# Autodesk Inventor assembly: SailAssembly
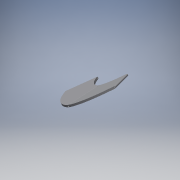
[picture p0: Inventor's stored thumbnail of the model, 180x180]
Saved by Autodesk Inventor 2018.3 (Build 223284000, 284)
## iProperties
Created: 2020-03-24
Part Number: SailAssembly
Document SubType Name: Assembly
Designer: ToreDenStore
Author: ToreDenStore
## Documents named in this file (2)
- C:\Users\ToreDenStore\Documents\Inventor\VAWT turbine sunfeather\SailAssembly.iam
- C:\Users\ToreDenStore\Documents\Inventor\VAWT turbine sunfeather\Sail.ipt
## Components (2 placed, 1 different names)
1. Sail:1 — Mate:1, Rotational:1
2. Sail:2 — Mate:1, Rotational:1
## Relationships (2: Mate 1, RevoluteJoint 1)
- Mate:1: Sail:1 ↔ Sail:2
- Rotational:1 [RevoluteJoint]: Sail:1 ↔ Sail:2
